# Autodesk Inventor assembly: motor_w_gear_MIR
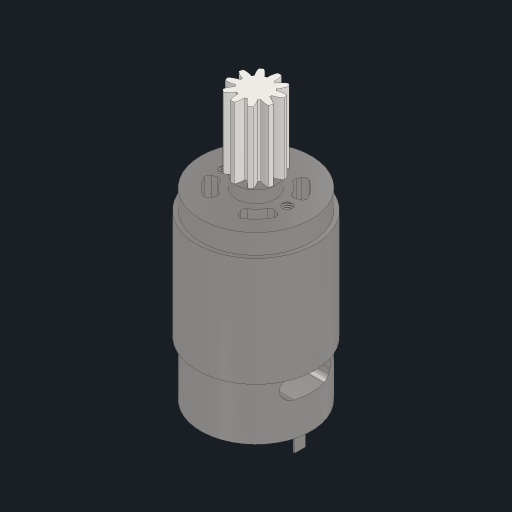
[picture p0: Inventor's stored thumbnail of the model, 512x512]
Saved by Autodesk Inventor 2023 (Build 270158000, 158)
## iProperties
Created: 2024-04-29
Part Number: motor_w_gear_MIR
Document SubType Name: Assembly
Designer: szymo
Mass: 122 g
Surface Area: 88.1762 cm^2
Volume: 30.6048 cm^3
TOTAL MASS: 0.0
Author: szymo
## Documents named in this file (3)
- D:\roboilo\robots\codename wafel - australia\3d_parts\rev4\motor_w_gear_MIR.iam
- D:\roboilo\robots\codename wafel - australia\3d_parts\rev4\rs390_MIR.ipt
- D:\roboilo\robots\codename wafel - australia\3d_parts\rev4\Design Accelerator\big_gear1_MIR.iam
## Components (2 placed, 2 different names)
1. rs390_MIR:1 — Mate:2, Mate:1
2. big_gear1_MIR:1 [sub-assembly] — Mate:2, Mate:1
## Relationships (2: Mate 2)
- Mate:2 (1 mm): rs390_MIR:1 ↔ big_gear1_MIR:1
- Mate:1: rs390_MIR:1 ↔ big_gear1_MIR:1
